# Autodesk Inventor assembly: stack
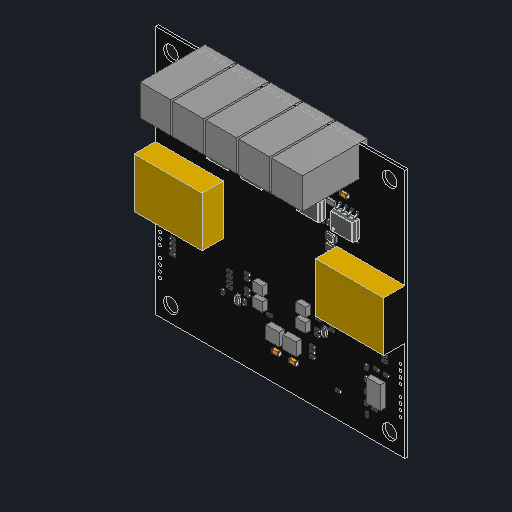
[picture p0: Inventor's stored thumbnail of the model, 512x512]
Saved by Autodesk Inventor 2023 (Build 270158000, 158)
## iProperties
Created: 2024-04-09
Part Number: stack
Document SubType Name: Assembly
Designer: szymo
Mass: 50 g
Surface Area: 207.755 cm^2
Volume: 9.85455 cm^3
Density: 5.0738 g/cm^3
Author: szymo
## Documents named in this file (3)
- D:\roboilo\robots\codename wafel - australia\3d_parts\rev4\stack.iam
- D:\roboilo\robots\codename wafel - australia\3d_parts\rev4\mcu.ipt
- D:\roboilo\robots\codename wafel - australia\3d_parts\rev4\Motor Driver.ipt
## Components (2 placed, 2 different names)
1. Motor Driver:1 — Mate:1, Flush:1, Flush:2
2. mcu:1 — Mate:1, Flush:1, Flush:2
## Relationships (3: Flush 2, Mate 1)
- Mate:1 (4.7 mm): Motor Driver:1 ↔ mcu:1
- Flush:1: Motor Driver:1 ↔ mcu:1
- Flush:2: Motor Driver:1 ↔ mcu:1
